# Autodesk Inventor assembly: Assembly
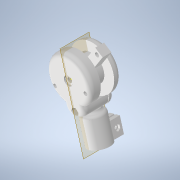
[picture p0: Inventor's stored thumbnail of the model, 180x180]
Saved by Autodesk Inventor 2021 (Build 250183000, 183)
## iProperties
Created: 2021-03-16
Part Number: Assembly
Document SubType Name: Assembly
Designer: Olivi
Author: Olivi
## Documents named in this file (6)
- C:\Users\Olivi\Universiteit Antwerpen\Plasma Robotics - General\3D parts\02 SCARA Robot\files\SCARA arm\Assembly.iam
- C:\Users\Olivi\Universiteit Antwerpen\Plasma Robotics - General\3D parts\02 SCARA Robot\files\SCARA arm\Motorconnection.ipt
- C:\Users\Olivi\Universiteit Antwerpen\Plasma Robotics - General\3D parts\02 SCARA Robot\files\SCARA arm\Motorshaft.ipt
- C:\Users\Olivi\Downloads\608zz-ball-bearing-1.snapshot.2\Ball_Bearing_608zz.ipt
- C:\Users\Olivi\Universiteit Antwerpen\Plasma Robotics - General\3D parts\02 SCARA Robot\files\SCARA arm\fixedpart.ipt
- C:\Users\Olivi\Universiteit Antwerpen\Plasma Robotics - General\3D parts\02 SCARA Robot\files\SCARA arm\Ball_Bearing_608zz.ipt
## Components (7 placed, 4 different names)
1. Motorconnection:1 — Insert:1
2. Motorshaft:1 — Insert:2, Insert:3
3. Ball_Bearing_608zz:1
4. Ball_Bearing_608zz:2
5. fixedpart:1
6. Ball_Bearing_608zz:3 — Insert:3
7. Ball_Bearing_608zz:4 — Insert:1, Insert:2
## Relationships (3: Insert 3)
- Insert:1: Motorconnection:1 ↔ Ball_Bearing_608zz:4
- Insert:2: Motorshaft:1 ↔ Ball_Bearing_608zz:4
- Insert:3: Motorshaft:1 ↔ Ball_Bearing_608zz:3
